# Autodesk Inventor assembly: Raspberry Pi 3
(part 2 of 2)
608. Raspberry Pi 3242_608
609. Raspberry Pi 3242_609
610. Raspberry Pi 3242_610
611. Raspberry Pi 3242_611
612. Raspberry Pi 3242_612
613. Raspberry Pi 3242_613
614. Raspberry Pi 3266_614
615. Raspberry Pi 3266_615
616. Raspberry Pi 3266_616
617. Raspberry Pi 3266_617
618. Raspberry Pi 3266_618
619. Raspberry Pi 3266_619
620. Raspberry Pi 3266_620
621. Raspberry Pi 3266_621
622. Raspberry Pi 3266_622
623. Raspberry Pi 3266_623
624. Raspberry Pi 3266_624
625. Raspberry Pi 3266_625
626. Raspberry Pi 3266_626
627. Raspberry Pi 3266_627
628. Raspberry Pi 3266_628
629. Raspberry Pi 3266_629
630. Raspberry Pi 3266_630
631. Raspberry Pi 3266_631
632. Raspberry Pi 3266_632
633. raspberry_pi_B_(RJ45)_633
